# Autodesk Inventor assembly: face
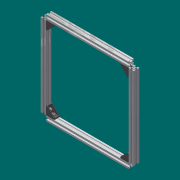
[picture p0: Inventor's stored thumbnail of the model, 180x180]
Saved by Autodesk Inventor 2016 SP1 (Build 200210100, 210)
## iProperties
Created: 2016-02-10
Part Number: face
Document SubType Name: Assembly
Designer: Sawaiz
Author: Sawaiz
## Documents named in this file (4)
- C:\Users\Sawaiz\OneDrive\projects\modularHodoscope\frame\face.iam
- C:\Users\Sawaiz\OneDrive\projects\modularHodoscope\frame\hfs5-2020Height.ipt
- C:\Users\Sawaiz\OneDrive\projects\modularHodoscope\frame\hfs5-2020Width.ipt
- C:\Users\Sawaiz\OneDrive\projects\modularHodoscope\hardware\angleBracket.iam
## Components (8 placed, 3 different names)
1. hfs5-2020Height:1 — Flush:1, Flush:2, Symmetry:1, Flush:8, Mate:6, Flush:14, Mate:7
2. hfs5-2020Height:2 — Flush:3, Symmetry:1, Flush:8, Mate:1, Flush:9, Mate:3, Flush:11, Symmetry:3
3. hfs5-2020Width:1 — Flush:1, Flush:6, Flush:7, Mate:2, Flush:10, Mate:5, Flush:13, Flush:15, Symmetry:2, Symmetry:3
4. hfs5-2020Width:2 — Flush:2, Flush:3, Flush:4, Flush:5, Mate:4, Flush:12, Mate:8, Symmetry:2
5. angleBracket:1 [sub-assembly] — Flush:6, Mate:5, Flush:13, Mate:6, Flush:14, Flush:15
6. angleBracket:2 [sub-assembly] — Flush:7, Mate:1, Flush:9, Mate:2, Flush:10
7. angleBracket:3 [sub-assembly] — Flush:4, Mate:3, Flush:11, Mate:4, Flush:12
8. angleBracket:4 [sub-assembly] — Flush:5, Mate:7, Mate:8
## Relationships (26: Flush 15, Mate 8, Symmetry 3)
- Flush:1: hfs5-2020Height:1 ↔ hfs5-2020Width:1
- Flush:2: hfs5-2020Height:1 ↔ hfs5-2020Width:2
- Flush:3: hfs5-2020Height:2 ↔ hfs5-2020Width:2
- Flush:4: hfs5-2020Width:2 ↔ angleBracket:3
- Flush:5: hfs5-2020Width:2 ↔ angleBracket:4
- Flush:6: hfs5-2020Width:1 ↔ angleBracket:1
- Flush:7: hfs5-2020Width:1 ↔ angleBracket:2
- Symmetry:1: hfs5-2020Height:1 ↔ hfs5-2020Height:2
- Flush:8: hfs5-2020Height:1 ↔ hfs5-2020Height:2
- Mate:1: hfs5-2020Height:2 ↔ angleBracket:2
- Flush:9: hfs5-2020Height:2 ↔ angleBracket:2
- Mate:2: hfs5-2020Width:1 ↔ angleBracket:2
- Flush:10: hfs5-2020Width:1 ↔ angleBracket:2
- Mate:3: hfs5-2020Height:2 ↔ angleBracket:3
- Flush:11: hfs5-2020Height:2 ↔ angleBracket:3
- Mate:4: hfs5-2020Width:2 ↔ angleBracket:3
- Flush:12: hfs5-2020Width:2 ↔ angleBracket:3
- Mate:5: hfs5-2020Width:1 ↔ angleBracket:1
- Flush:13: hfs5-2020Width:1 ↔ angleBracket:1
- Mate:6: hfs5-2020Height:1 ↔ angleBracket:1
- Flush:14: hfs5-2020Height:1 ↔ angleBracket:1
- Flush:15: hfs5-2020Width:1 ↔ angleBracket:1
- Mate:7: hfs5-2020Height:1 ↔ angleBracket:4
- Mate:8: hfs5-2020Width:2 ↔ angleBracket:4
- Symmetry:2: hfs5-2020Width:1 ↔ hfs5-2020Width:2
- Symmetry:3: hfs5-2020Height:2 ↔ hfs5-2020Width:1
